# Autodesk Inventor assembly: small pulley
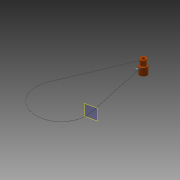
[picture p0: Inventor's stored thumbnail of the model, 180x180]
Saved by Autodesk Inventor 2013 (Build 170138000, 138)
## iProperties
Created: 2013-10-18
Part Number: small pulley
Document SubType Name: Assembly
Designer: employee
Author: employee
## Documents named in this file (4)
- C:\Users\employee\Desktop\new wally\small pulley.iam
- C:\Users\employee\Desktop\new wally\xy pulley.ipt
- C:\Users\employee\Desktop\new wally\string.ipt
- C:\Users\employee\Desktop\new wally\M3x10.ipt
## Components (3 placed, 3 different names)
1. xy pulley:1 — Mate:1, Mate:2, Mate:3, Mate:4
2. string:1 — Mate:1, Mate:2
3. M3x10:1 — Mate:3, Mate:4
## Relationships (4: Mate 4)
- Mate:1: xy pulley:1 ↔ string:1
- Mate:2 (5 mm): xy pulley:1 ↔ string:1
- Mate:3 (2 mm): xy pulley:1 ↔ M3x10:1
- Mate:4: xy pulley:1 ↔ M3x10:1
